# Autodesk Inventor assembly: KVA Assembly Automation
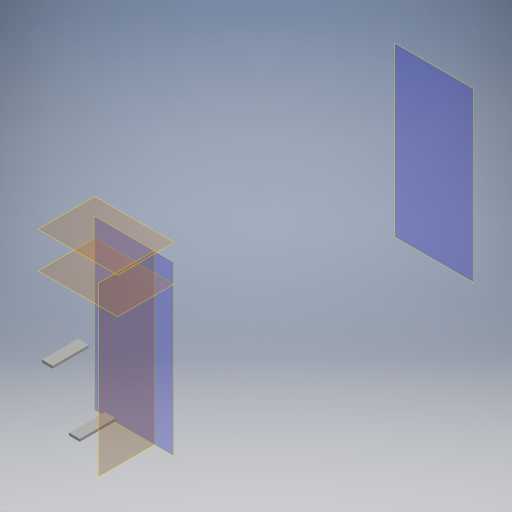
[picture p0: Inventor's stored thumbnail of the model, 512x512]
Saved by Autodesk Inventor 2024.2 (Build 282272000, 272)
## iProperties
Created: 2024-09-04
Part Number: KVA Assembly Automation
Document SubType Name: Assembly
Designer: TiffanyHayden
Author: TiffanyHayden
## Documents named in this file (2)
- C:\Users\TiffanyHayden\Documents\GitHub\KVA\Assemblies in Autodesk Inventor - Planning for Automation\KVA Assembly Automation.iam
- C:\Blog\Assets\ATQ-36-120-N.ipt
## Components (2 placed, 1 different names)
1. ATQ-36-120-N:1
2. ATQ-36-120-N:2
## Relationships (6: Flush 6)
- Flush:6 (-7620 mm)
- Flush:7
- Flush:8 (25400 mm)
- Flush:9 (3048 mm)
- Flush:10
- Flush:11
## Named parameters: OAL = 25400 mm, GATE_LOCATION = 7620 mm, HEIGHT = 3048 mm
